# Autodesk Inventor assembly: H12700A
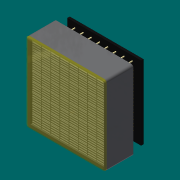
[picture p0: Inventor's stored thumbnail of the model, 180x180]
Saved by Autodesk Inventor 2016 SP1 (Build 200210100, 210)
## iProperties
Created: 2015-10-20
Part Number: H12700A
Document SubType Name: Assembly
Designer: Sawaiz
Author: Sawaiz
## Documents named in this file (4)
- C:\Users\sawai\OneDrive\projects\modularRICH\H12700A\H12700A.iam
- C:\Users\sawai\OneDrive\projects\modularRICH\H12700A\H12700A.ipt
- C:\Users\sawai\OneDrive\projects\modularRICH\H12700A\headderPanel.ipt
- C:\Users\sawai\OneDrive\projects\modularRICH\H12700A\2x18header2mm.ipt
## Components (6 placed, 3 different names)
1. H12700A:1 — Mate:1, Flush:1, Flush:2
2. headderPanel:1 — Mate:1, Flush:1, Mate:2, Angle:1, Mate:3, Flush:2
3. 2x18header2mm:1 — Mate:2, Angle:1, Mate:3
4. 2x18header2mm:2
5. 2x18header2mm:3
6. 2x18header2mm:4
## Component patterns: (4 elements, first: 2x18header2mm:1)
## Relationships (6: Mate 3, Flush 2, Angle 1)
- Mate:1 (-27.4 mm): H12700A:1 ↔ headderPanel:1
- Flush:1 (1.75 mm): H12700A:1 ↔ headderPanel:1
- Mate:2: headderPanel:1 ↔ 2x18header2mm:1
- Angle:1 (0 deg): headderPanel:1 ↔ 2x18header2mm:1
- Mate:3: headderPanel:1 ↔ 2x18header2mm:1
- Flush:2 (1.75 mm): H12700A:1 ↔ headderPanel:1
